# Autodesk Inventor assembly: Backpack
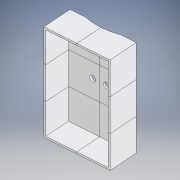
[picture p0: Inventor's stored thumbnail of the model, 180x180]
Saved by Autodesk Inventor 2017 SP1 (Build 210196100, 196)
## iProperties
Created: 2017-09-05
Part Number: Backpack
Document SubType Name: Assembly
Designer: Zach
Author: Zach
## Documents named in this file (5)
- C:\Users\Zach\Documents\GitHub\tr1\src\Body\Chest Assembly\Backpack Assembly\Backpack.iam
- C:\Users\Zach\Documents\GitHub\tr1\src\Body\Chest Assembly\Backpack Assembly\BP001.ipt
- C:\Users\Zach\Documents\GitHub\tr1\src\Body\Chest Assembly\Backpack Assembly\BP002.ipt
- C:\Users\Zach\Documents\GitHub\tr1\src\Body\Chest Assembly\Backpack Assembly\BP003.ipt
- C:\Users\Zach\Documents\GitHub\tr1\src\Body\Chest Assembly\Backpack Assembly\BP004.ipt
## Components (6 placed, 4 different names)
1. BP001:1 — Mate:1, Mate:2, Mate:3, Mate:4, Flush:1, Flush:3, Flush:7, Flush:12
2. BP001:2 — Mate:7, Flush:8, Mate:10, Flush:10, Mate:12
3. BP002:1 — Mate:1, Mate:2, Flush:3, Flush:7, Mate:9, Flush:13, Mate:11
4. BP002:2 — Mate:7, Mate:8, Flush:8, Flush:11, Mate:12
5. BP003:1 — Mate:3, Mate:4, Flush:1, Mate:8, Flush:9, Flush:11, Flush:12
6. BP004:1 — Mate:9, Mate:10, Flush:9, Flush:10, Flush:13, Mate:11
## Relationships (19: Mate 10, Flush 9)
- Mate:1: BP001:1 ↔ BP002:1
- Mate:2: BP001:1 ↔ BP002:1
- Mate:3: BP001:1 ↔ BP003:1
- Mate:4: BP001:1 ↔ BP003:1
- Flush:1: BP001:1 ↔ BP003:1
- Flush:3: BP001:1 ↔ BP002:1
- Flush:7: BP001:1 ↔ BP002:1
- Mate:7: BP001:2 ↔ BP002:2
- Mate:8: BP002:2 ↔ BP003:1
- Flush:8: BP001:2 ↔ BP002:2
- Mate:9: BP002:1 ↔ BP004:1
- Mate:10: BP001:2 ↔ BP004:1
- Flush:9: BP003:1 ↔ BP004:1
- Flush:10: BP001:2 ↔ BP004:1
- Flush:11: BP002:2 ↔ BP003:1
- Flush:12: BP001:1 ↔ BP003:1
- Flush:13: BP002:1 ↔ BP004:1
- Mate:11: BP002:1 ↔ BP004:1
- Mate:12: BP001:2 ↔ BP002:2
